# Autodesk Inventor assembly: bett_V1_sitzbank_mit_deckel
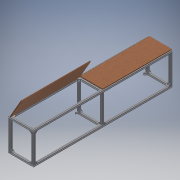
[picture p0: Inventor's stored thumbnail of the model, 180x180]
Saved by Autodesk Inventor 2018 (Build 220112000, 112)
## iProperties
Created: 2020-04-13
Part Number: bett_V1_sitzbank_mit_deckel
Material: Generisch
Document SubType Name: Assembly
Designer: wepet
Author: wepet
## Documents named in this file (3)
- C:\Users\wepet\Downloads\anhaenger\current\details\bett\bett_V1\bett_V1.iam
- C:\Users\wepet\Downloads\anhaenger\current\details\bett\bett_V1\bett_V1_teil1_sitzbank.iam
- C:\Users\wepet\Downloads\anhaenger\current\details\bett\bett_V1\bett_V1_teil2_deckplatte.ipt
## Components (3 placed, 2 different names)
1. bett_V1_teil1_sitzbank:1 [sub-assembly] — Drehbar:1, Drehbar:2, Passend:1, Passend:2, Passend:3
2. bett_V1_teil2_deckplatte:1 — Drehbar:1
3. bett_V1_teil2_deckplatte:2 — Drehbar:2
## Relationships (5: Mate 3, RevoluteJoint 2)
- Drehbar:1 [RevoluteJoint]: bett_V1_teil1_sitzbank:1 ↔ bett_V1_teil2_deckplatte:1
- Drehbar:2 [RevoluteJoint]: bett_V1_teil1_sitzbank:1 ↔ bett_V1_teil2_deckplatte:2
- Passend:1 [Mate]: bett_V1_teil1_sitzbank:1
- Passend:2 [Mate]: bett_V1_teil1_sitzbank:1
- Passend:3 [Mate]: bett_V1_teil1_sitzbank:1
